# Autodesk Inventor assembly: 240710_case
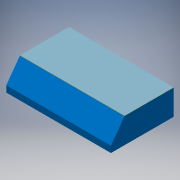
[picture p0: Inventor's stored thumbnail of the model, 180x180]
Saved by Autodesk Inventor 2016 (Build 200138000, 138)
## iProperties
Created: 2024-07-10
Part Number: 240710_case
Material: 일반
Document SubType Name: Assembly
Designer: pc
Author: pc
## Documents named in this file (3)
- D:\CAD_HCH\240710\240710_case.iam
- D:\CAD_HCH\240710\240710_part2.ipt
- D:\CAD_HCH\240710\240710_part3.ipt
## Components (2 placed, 2 different names)
1. 240710_part2:1 — 메이트:1, 플러쉬:1, 플러쉬:2
2. 240710_part3:1 — 메이트:1, 플러쉬:1, 플러쉬:2
## Relationships (3: Flush 2, Mate 1)
- 메이트:1 [Mate]: 240710_part2:1 ↔ 240710_part3:1
- 플러쉬:1 [Flush]: 240710_part2:1 ↔ 240710_part3:1
- 플러쉬:2 [Flush]: 240710_part2:1 ↔ 240710_part3:1
